# Autodesk Inventor assembly: Drone
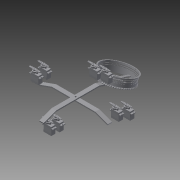
[picture p0: Inventor's stored thumbnail of the model, 180x180]
Saved by Autodesk Inventor 2015 (Build 190159000, 159)
## iProperties
Created: 2015-06-16
Part Number: Drone
Document SubType Name: Assembly
Designer: david_000
Author: david_000
## Documents named in this file (4)
- J:\Drone\Drone.iam
- J:\Drone\Frame.ipt
- J:\Drone\FanChais.iam
- J:\Drone\Imported Components\MicroServo9g\MicroServo9g.iam
## Components (11 placed, 3 different names)
1. Frame:1 — Mate:1, Angle:1, Tangent:1
2. Frame:2 — Mate:1, Angle:1, Tangent:1, Mate:2
3. FanChais:1 [sub-assembly] — Mate:2
4. MicroServo9g:1 [sub-assembly]
5. MicroServo9g:2 [sub-assembly]
6. MicroServo9g:3 [sub-assembly]
7. MicroServo9g:4 [sub-assembly]
8. MicroServo9g:5 [sub-assembly]
9. MicroServo9g:6 [sub-assembly]
10. MicroServo9g:7 [sub-assembly]
11. MicroServo9g:8 [sub-assembly]
## Relationships (4: Mate 2, Angle 1, Tangent 1)
- Mate:1: Frame:1 ↔ Frame:2
- Angle:1 (90 deg): Frame:1 ↔ Frame:2
- Tangent:1: Frame:1 ↔ Frame:2
- Mate:2: Frame:2 ↔ FanChais:1
